# Autodesk Inventor assembly: motormodul
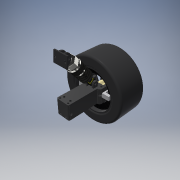
[picture p0: Inventor's stored thumbnail of the model, 180x180]
Saved by Autodesk Inventor 2016 (Build 200138000, 138)
## iProperties
Created: 2016-11-21
Part Number: motormodul
Document SubType Name: Assembly
Designer: Juraj
Author: Juraj
## Documents named in this file (8)
- C:\Users\Juraj\Documents\GitHub\Robot6x6\Terrenny robot CAD\motormodul.iam
- C:\Users\Juraj\Documents\GitHub\Robot6x6\Terrenny robot CAD\uchyt_motor\motor.iam
- C:\Users\Juraj\Documents\GitHub\Robot6x6\Terrenny robot CAD\spojka_oska_koleso.ipt
- C:\Users\Juraj\Documents\GitHub\Robot6x6\Terrenny robot CAD\uchytpruzina.ipt
- C:\Users\Juraj\Documents\GitHub\Robot6x6\Terrenny robot CAD\pruzina\pruzina.iam
- C:\Users\Juraj\Documents\GitHub\Robot6x6\Terrenny robot CAD\koleso\koleso.iam
- C:\Users\Juraj\Documents\GitHub\Robot6x6\Terrenny robot CAD\otackomer_new.ipt
- C:\Users\Juraj\Desktop\otackomer.ipt
## Components (8 placed, 7 different names)
1. motor:1 [sub-assembly] — Insert:2, Insert:4, Mate:1, Mate:2, Mate:3, Mate:4, Mate:5, Mate:7, Mate:8
2. spojka_oska_koleso:1 — Insert:2, Insert:5
3. uchytpruzina:1 — Insert:3
4. pruzina:1 [sub-assembly] — Insert:3, Insert:4
5. koleso:1 [sub-assembly] — Insert:5, Insert:6
6. otackomer_new:1 — Insert:6
7. otackomer:1 — Mate:4, Mate:5
8. otackomer:2 — Mate:7, Mate:8
## Relationships (12: Mate 7, Insert 5)
- Insert:2: motor:1 ↔ spojka_oska_koleso:1
- Insert:3 (0.45 mm): uchytpruzina:1 ↔ pruzina:1
- Insert:4 (1.6 mm): motor:1 ↔ pruzina:1
- Insert:5: spojka_oska_koleso:1 ↔ koleso:1
- Insert:6 (15 mm): koleso:1 ↔ otackomer_new:1
- Mate:1: motor:1
- Mate:2: motor:1
- Mate:3: motor:1
- Mate:4: motor:1 ↔ otackomer:1
- Mate:5 (0.567 mm): motor:1 ↔ otackomer:1
- Mate:7: motor:1 ↔ otackomer:2
- Mate:8: motor:1 ↔ otackomer:2
